# Autodesk Inventor assembly: B Drive
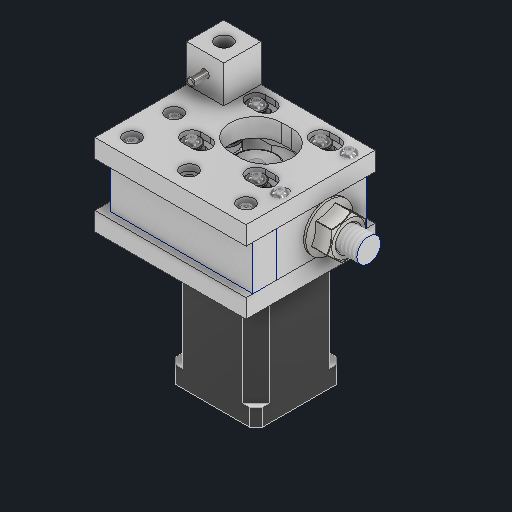
[picture p0: Inventor's stored thumbnail of the model, 512x512]
Saved by Autodesk Inventor 2025.1 (Build 291241020, 241B)
## iProperties
Created: 2025-05-09
Part Number: B Drive
Document SubType Name: Assembly
Designer: AdminForWorker
Title: B Drive
Author: AdminForWorker
## Documents named in this file (9)
- C:\Users\Joshua Eah\Documents\Voron 0.2\CAD\Master Assembly\Motion\AB Drives\B Drive.iam
- C:\Users\Joshua Eah\Documents\Voron 0.2\CAD\Machined Parts\AB Drives\B Drive\B Drive Assembly.iam
- C:\Users\Joshua Eah\Documents\Voron 0.2\CAD\Master Assembly\Motion\AB Drives\Motor Assembly.iam
- C:\Users\Joshua Eah\Documents\Voron 0.2\CAD\Master Assembly\Hardware\M3x10 BHCS.ipt
- C:\Users\Joshua Eah\Documents\Voron 0.2\CAD\Master Assembly\Hardware\M3x35 BHCS.ipt
- C:\Users\Joshua Eah\Documents\Voron 0.2\CAD\Master Assembly\Hardware\M3x30 BHCS.ipt
- C:\Users\Joshua Eah\Documents\Voron 0.2\CAD\Master Assembly\F623 Stack.iam
- C:\Users\Joshua Eah\Documents\Voron 0.2\CAD\Master Assembly\Hardware\M3 Hexnut.ipt
- C:\Users\Joshua Eah\Documents\Voron 0.2\CAD\Master Assembly\Hardware\M3_Washer.ipt
## Components (23 placed, 8 different names)
1. B Drive Assembly:1 [sub-assembly] — Mate:3
2. Motor Assembly:1 [sub-assembly] — Mate:3
3. M3x10 BHCS:1
4. M3x35 BHCS:1
5. M3x35 BHCS:2
6. M3x35 BHCS:3
7. M3x35 BHCS:4
8. M3x35 BHCS:5
9. M3x35 BHCS:6
10. M3x35 BHCS:7
11. M3x35 BHCS:8
12. M3x30 BHCS:1
13. M3x30 BHCS:2
14. F623 Stack:1 [sub-assembly]
15. F623 Stack:2 [sub-assembly]
16. F623 Stack:3 [sub-assembly]
17. M3 Hexnut:1
18. M3 Hexnut:2
19. M3 Hexnut:3
20. M3 Washer (1):1
21. M3 Washer (1):2
22. M3 Washer (1):3
23. M3 Washer (1):4
## Relationships (5: Mate 3, Insert 2)
- [Insert]: B Drive Assembly:1 ↔ M3x10 BHCS:1
- [Insert]: B Drive Assembly:1 ↔ M3x35 BHCS:6
- [Mate]: Motor Assembly:1 ↔ M3x35 BHCS:7
- [Mate]: Motor Assembly:1 ↔ M3x35 BHCS:8
- Mate:3: B Drive Assembly:1 ↔ Motor Assembly:1
